# Autodesk Inventor assembly: Assembly_Huawei_P30_Scanninglens
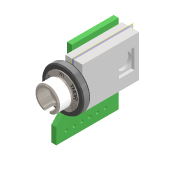
[picture p0: Inventor's stored thumbnail of the model, 180x180]
Saved by Autodesk Inventor 2022 (Build 260153000, 153)
## iProperties
Created: 2022-12-14
Part Number: Assembly_Huawei_P30_Scanninglens
Document SubType Name: Assembly
Designer: diederichbenedict
Author: diederichbenedict
## Documents named in this file (5)
- C:\Users\diederichbenedict\Dropbox\Dokumente\Promotion\PROJECTS\HoLiSheet\INVENTOR\Assembly_Huawei_P30_Scanninglens.iam
- C:\Users\diederichbenedict\Dropbox\Dokumente\Promotion\PROJECTS\HoLiSheet\INVENTOR\00_huawei_p30_Objectivelensassembly.ipt
- C:\Users\diederichbenedict\Dropbox\Dokumente\Promotion\PROJECTS\HoLiSheet\INVENTOR\00_Huawei_P30_Lens_Adapterpcb.ipt
- C:\Users\diederichbenedict\Dropbox\Dokumente\Promotion\PROJECTS\HoLiSheet\INVENTOR\00_SMAConnector_fiber copy.ipt
- C:\Users\diederichbenedict\Dropbox\Dokumente\Promotion\PROJECTS\HoLiSheet\INVENTOR\HoLiSheet.ipt
## Components (4 placed, 4 different names)
1. 00_huawei_p30_Objectivelensassembly:1 — Fluchtend:1, Einfügen:1
2. 00_Huawei_P30_Lens_Adapterpcb:1 — Fluchtend:1, Fluchtend:2, Fluchtend:3, Fluchtend:4
3. 00_SMAConnector_fiber copy:1 — Einfügen:1, Winkel:1
4. HoLiSheet:1 — Fluchtend:2, Fluchtend:3, Fluchtend:4
## Relationships (6: Flush 4, Insert 1, Angle 1)
- Fluchtend:1 [Flush]: 00_huawei_p30_Objectivelensassembly:1 ↔ 00_Huawei_P30_Lens_Adapterpcb:1
- Einfügen:1 [Insert] (-1 mm): 00_huawei_p30_Objectivelensassembly:1 ↔ 00_SMAConnector_fiber copy:1
- Winkel:1 [Angle] (0 deg): 00_SMAConnector_fiber copy:1
- Fluchtend:2 [Flush]: 00_Huawei_P30_Lens_Adapterpcb:1 ↔ HoLiSheet:1
- Fluchtend:3 [Flush]: 00_Huawei_P30_Lens_Adapterpcb:1 ↔ HoLiSheet:1
- Fluchtend:4 [Flush]: 00_Huawei_P30_Lens_Adapterpcb:1 ↔ HoLiSheet:1
